# Autodesk Inventor assembly: Assembly Plate Assembly
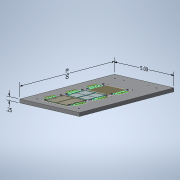
[picture p0: Inventor's stored thumbnail of the model, 180x180]
Saved by Autodesk Inventor 2022 (Build 260153000, 153)
## iProperties
Created: 2021-01-11
Part Number: Assembly Plate Assembly
Document SubType Name: Assembly
Designer: caleb
Author: caleb
## Documents named in this file (5)
- C:\Users\Caleb\Desktop\nebraska-silicon-lab\Hardware\ETL\Module Assembly\Assembly Plate\Assembly Plate Assembly.iam
- C:\Users\Caleb\Desktop\nebraska-silicon-lab\Hardware\ETL\Module Assembly\Assembly Plate\Assembly Plate.ipt
- C:\Users\Caleb\Desktop\nebraska-silicon-lab\Hardware\ETL\modules\tdr\F10110887--_1-MODULE_ CMS2 ETL_ FULL DBL-SENSOR MOUNTED ASSY.iam
- C:\Users\Caleb\Desktop\nebraska-silicon-lab\Hardware\ETL\modules\tdr\Module without cover.iam
- C:\Users\Caleb\Desktop\nebraska-silicon-lab\Hardware\ETL\modules\tdr\Module baseplate only.iam
## Components (4 placed, 4 different names)
1. Assembly Plate:1 — Mate:1, Angle:1, Mate:2, Angle:2, Mate:3, Angle:3
2. F10110887--_1-MODULE_ CMS2 ETL_ FULL DBL-SENSOR MOUNTED ASSY:1 [sub-assembly] — Mate:1, Angle:1
3. Module without cover:1 [sub-assembly] — Mate:2, Angle:2
4. Module baseplate only:1 [sub-assembly] — Mate:3, Angle:3
## Relationships (6: Mate 3, Angle 3)
- Mate:1: Assembly Plate:1 ↔ F10110887--_1-MODULE_ CMS2 ETL_ FULL DBL-SENSOR MOUNTED ASSY:1
- Angle:1 (0 deg): Assembly Plate:1 ↔ F10110887--_1-MODULE_ CMS2 ETL_ FULL DBL-SENSOR MOUNTED ASSY:1
- Mate:2: Assembly Plate:1 ↔ Module without cover:1
- Angle:2 (0 deg): Assembly Plate:1 ↔ Module without cover:1
- Mate:3: Assembly Plate:1 ↔ Module baseplate only:1
- Angle:3 (0 deg): Assembly Plate:1 ↔ Module baseplate only:1
